# Autodesk Inventor assembly: Leg_joint_roll_yaw
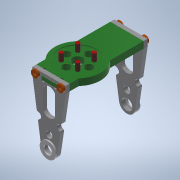
[picture p0: Inventor's stored thumbnail of the model, 180x180]
Saved by Autodesk Inventor 2020 (Build 240168000, 168)
## iProperties
Created: 2016-05-01
Part Number: Leg_joint_roll_yaw
Document SubType Name: Assembly
Designer: hiroaki
Mass: 101.489 g
Surface Area: 218.083 cm^2
Volume: 17.9148 cm^3
Density: 5.6651 g/cm^3
Author: hiroaki
## Documents named in this file (6)
- C:\Users\Masato\Documents\Inventor\CIT Brains_Inventor\OpenPlatform_ver3_0\LowerBody\Leg_joit\Leg_joint_roll_yaw.iam
- C:\Users\Masato\Documents\Inventor\CIT Brains_Inventor\OpenPlatform_ver3_0\LowerBody\Leg_joit\Leg_joint_yaw_frame.ipt
- C:\Users\Masato\Documents\Inventor\CIT Brains_Inventor\OpenPlatform_ver3_0\Ready_Made\Screw\M3-10.ipt
- C:\Users\Masato\Documents\Inventor\CIT Brains_Inventor\OpenPlatform_ver3_0\Ready_Made\Screw\M3-6.ipt
- C:\Users\Masato\Documents\Inventor\CIT Brains_Inventor\OpenPlatform_ver3_0\LowerBody\Leg_joit\Leg_joint_slider_frame.ipt
- C:\Users\Masato\Documents\Inventor\CIT Brains_Inventor\OpenPlatform_ver3_0\Ready_Made\TT-0612-10.ipt
## Components (13 placed, 5 different names)
1. Leg_joint_yaw_frame:1 — 挿入:53, 挿入:54, 挿入:55, 挿入:56, 挿入:66, 挿入:67, 挿入:71, 挿入:72
2. M3-10:1 — 挿入:53
3. M3-10:2 — 挿入:54
4. M3-10:3 — 挿入:55
5. M3-10:4 — 挿入:56
6. M3-6:1 — 挿入:74
7. M3-6:2 — 挿入:73
8. M3-6:3 — 挿入:68
9. M3-6:4 — 挿入:69
10. Leg_joint_slider_frame:1 — 挿入:66, 挿入:67, 挿入:68, 挿入:69, 挿入:76
11. Leg_joint_slider_frame:2 — 挿入:71, 挿入:72, 挿入:73, 挿入:74, 挿入:75
12. TT-0612-10:1 — 挿入:75
13. TT-0612-10:2 — 挿入:76
## Relationships (14: Insert 14)
- 挿入:53 [Insert]: Leg_joint_yaw_frame:1 ↔ M3-10:1
- 挿入:54 [Insert]: Leg_joint_yaw_frame:1 ↔ M3-10:2
- 挿入:55 [Insert]: Leg_joint_yaw_frame:1 ↔ M3-10:3
- 挿入:56 [Insert]: Leg_joint_yaw_frame:1 ↔ M3-10:4
- 挿入:66 [Insert]: Leg_joint_yaw_frame:1 ↔ Leg_joint_slider_frame:1
- 挿入:67 [Insert]: Leg_joint_yaw_frame:1 ↔ Leg_joint_slider_frame:1
- 挿入:68 [Insert]: M3-6:3 ↔ Leg_joint_slider_frame:1
- 挿入:69 [Insert]: M3-6:4 ↔ Leg_joint_slider_frame:1
- 挿入:71 [Insert]: Leg_joint_yaw_frame:1 ↔ Leg_joint_slider_frame:2
- 挿入:72 [Insert]: Leg_joint_yaw_frame:1 ↔ Leg_joint_slider_frame:2
- 挿入:73 [Insert]: M3-6:2 ↔ Leg_joint_slider_frame:2
- 挿入:74 [Insert]: M3-6:1 ↔ Leg_joint_slider_frame:2
- 挿入:75 [Insert]: Leg_joint_slider_frame:2 ↔ TT-0612-10:1
- 挿入:76 [Insert]: Leg_joint_slider_frame:1 ↔ TT-0612-10:2
